# Autodesk Inventor assembly: Y-Carriage_LM3037
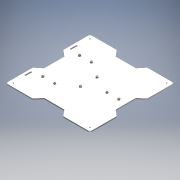
[picture p0: Inventor's stored thumbnail of the model, 180x180]
Saved by Autodesk Inventor 2020.2 (Build 242310000, 310)
## iProperties
Created: 2020-04-10
Part Number: Y-Carriage_LM3037
Document SubType Name: Assembly
Designer: rah75
Author: rah75
## Documents named in this file (10)
- C:\Users\rah75\Documents\GitHub\LETU-Maker\CAD\Autodesk Inventor\Base_3001-5999\Y-Carriage\Assemblies\Y-Carriage_LM3037.iam
- C:\Users\rah75\Documents\GitHub\LETU-Maker\CAD\Autodesk Inventor\Base_3001-5999\Y-Carriage\Fabricated_Parts\Y-Carriage_Plate_LM3033.ipt
- C:\Users\rah75\Documents\GitHub\LETU-Maker\CAD\Autodesk Inventor\Base_3001-5999\Y-Carriage\Printed_Parts\Y-Carriage_Belt_Mount_LM3035.ipt
- C:\Users\rah75\Documents\GitHub\LETU-Maker\CAD\Autodesk Inventor\Base_3001-5999\Y-Carriage\Printed_Parts\Y-Carriage_Belt_Clamp_LM3036.ipt
- C:\Users\rah75\Documents\GitHub\LETU-Maker\CAD\Autodesk Inventor\Base_3001-5999\Y-Carriage\Printed_Parts\Y-Carriage_Bearing_Mount_LM3034.ipt
- C:\Users\rah75\Documents\GitHub\LETU-Maker\CAD\Autodesk Inventor\Stock_Components_1001-2999\Fasteners\Nuts\heat_insert_m3_LM1017.ipt
- C:\Users\rah75\Documents\GitHub\LETU-Maker\CAD\Autodesk Inventor\Stock_Components_1001-2999\Power_Transmission\Bearings\linear_bearing_8x15mm_LM1031.ipt
- C:\Users\rah75\Documents\GitHub\LETU-Maker\CAD\Autodesk Inventor\Stock_Components_1001-2999\Fasteners\Screws\SHCS_m3x10_LM1015.ipt
- C:\Users\rah75\Documents\GitHub\LETU-Maker\CAD\Autodesk Inventor\Stock_Components_1001-2999\Fasteners\Washers_Spacers\washer_m3_LM1001.ipt
- C:\Users\rah75\Documents\GitHub\LETU-Maker\CAD\Autodesk Inventor\Stock_Components_1001-2999\Fasteners\Nuts\hex_nut_m3_LM1019.ipt
## Components (46 placed, 9 different names)
1. Y-Carriage_Plate_LM3033:1 — Insert:1, Insert:2, Insert:3, Insert:10, Mate:1, Insert:28, Insert:29, Insert:30, Insert:31, Insert:32, Insert:33, Insert:34, Insert:35
2. Y-Carriage_Belt_Mount_LM3035:1 — Insert:4, Insert:5, Insert:6, Insert:7, Insert:8, Insert:9
3. Y-Carriage_Belt_Clamp_LM3036:1 — Insert:12, Mate:3, Insert:36, Insert:37
4. Y-Carriage_Bearing_Mount_LM3034:1 — Insert:2, Insert:13, Insert:44, Insert:45
5. Y-Carriage_Bearing_Mount_LM3034:2 — Insert:3, Insert:15, Insert:40, Insert:41
6. Y-Carriage_Bearing_Mount_LM3034:3 — Insert:1, Insert:14, Insert:42, Insert:43
7. Y-Carriage_Belt_Clamp_LM3036:2 — Insert:11, Mate:2, Insert:38, Insert:39
8. heat_insert_m3_LM1017:1 — Insert:7, Insert:12
9. heat_insert_m3_LM1017:2 — Insert:5, Mate:2
10. heat_insert_m3_LM1017:3 — Insert:6, Mate:3
11. heat_insert_m3_LM1017:4 — Insert:9, Mate:1
12. heat_insert_m3_LM1017:5 — Insert:4, Insert:11
13. heat_insert_m3_LM1017:6 — Insert:8, Insert:10
14. linear_bearing_8x15mm_LM1031:1 — Insert:15
15. linear_bearing_8x15mm_LM1031:2 — Insert:14
16. linear_bearing_8x15mm_LM1031:3 — Insert:13
17. SHCS_m3x10_LM1015:1 — Insert:19
18. SHCS_m3x10_LM1015:2 — Insert:24
19. SHCS_m3x10_LM1015:3 — Insert:23
20. SHCS_m3x10_LM1015:4 — Insert:22
21. SHCS_m3x10_LM1015:5 — Insert:17
22. SHCS_m3x10_LM1015:6 — Insert:18
23. SHCS_m3x10_LM1015:7 — Insert:16
24. SHCS_m3x10_LM1015:8 — Insert:20
25. SHCS_m3x10_LM1015:9 — Insert:21
26. SHCS_m3x10_LM1015:10 — Insert:27
27. SHCS_m3x10_LM1015:11 — Insert:26
28. SHCS_m3x10_LM1015:12 — Insert:25
29. washer_m3_LM1001:1 — Insert:21, Insert:33
30. washer_m3_LM1001:2 — Insert:18, Insert:37
31. washer_m3_LM1001:3 — Insert:20, Insert:34
32. washer_m3_LM1001:4 — Insert:22, Insert:32
33. washer_m3_LM1001:5 — Insert:27, Insert:28
34. washer_m3_LM1001:6 — Insert:26, Insert:35
35. washer_m3_LM1001:7 — Insert:23, Insert:38
36. washer_m3_LM1001:8 — Insert:25, Insert:39
37. washer_m3_LM1001:9 — Insert:24, Insert:29
38. washer_m3_LM1001:10 — Insert:19, Insert:30
39. washer_m3_LM1001:11 — Insert:17, Insert:31
40. washer_m3_LM1001:12 — Insert:16, Insert:36
41. hex_nut_m3_LM1019:1 — Insert:40
42. hex_nut_m3_LM1019:2 — Insert:43
43. hex_nut_m3_LM1019:3 — Insert:44
44. hex_nut_m3_LM1019:4 — Insert:45
45. hex_nut_m3_LM1019:5 — Insert:42
46. hex_nut_m3_LM1019:6 — Insert:41
## Relationships (48: Insert 45, Mate 3)
- Insert:1: Y-Carriage_Plate_LM3033:1 ↔ Y-Carriage_Bearing_Mount_LM3034:3
- Insert:2: Y-Carriage_Plate_LM3033:1 ↔ Y-Carriage_Bearing_Mount_LM3034:1
- Insert:3: Y-Carriage_Plate_LM3033:1 ↔ Y-Carriage_Bearing_Mount_LM3034:2
- Insert:4: Y-Carriage_Belt_Mount_LM3035:1 ↔ heat_insert_m3_LM1017:5
- Insert:5: Y-Carriage_Belt_Mount_LM3035:1 ↔ heat_insert_m3_LM1017:2
- Insert:6: Y-Carriage_Belt_Mount_LM3035:1 ↔ heat_insert_m3_LM1017:3
- Insert:7: Y-Carriage_Belt_Mount_LM3035:1 ↔ heat_insert_m3_LM1017:1
- Insert:8: Y-Carriage_Belt_Mount_LM3035:1 ↔ heat_insert_m3_LM1017:6
- Insert:9: Y-Carriage_Belt_Mount_LM3035:1 ↔ heat_insert_m3_LM1017:4
- Insert:10: Y-Carriage_Plate_LM3033:1 ↔ heat_insert_m3_LM1017:6
- Mate:1: Y-Carriage_Plate_LM3033:1 ↔ heat_insert_m3_LM1017:4
- Insert:11: Y-Carriage_Belt_Clamp_LM3036:2 ↔ heat_insert_m3_LM1017:5
- Insert:12: Y-Carriage_Belt_Clamp_LM3036:1 ↔ heat_insert_m3_LM1017:1
- Mate:2: Y-Carriage_Belt_Clamp_LM3036:2 ↔ heat_insert_m3_LM1017:2
- Mate:3: Y-Carriage_Belt_Clamp_LM3036:1 ↔ heat_insert_m3_LM1017:3
- Insert:13: Y-Carriage_Bearing_Mount_LM3034:1 ↔ linear_bearing_8x15mm_LM1031:3
- Insert:14: Y-Carriage_Bearing_Mount_LM3034:3 ↔ linear_bearing_8x15mm_LM1031:2
- Insert:15: Y-Carriage_Bearing_Mount_LM3034:2 ↔ linear_bearing_8x15mm_LM1031:1
- Insert:16: SHCS_m3x10_LM1015:7 ↔ washer_m3_LM1001:12
- Insert:17: SHCS_m3x10_LM1015:5 ↔ washer_m3_LM1001:11
- Insert:18: SHCS_m3x10_LM1015:6 ↔ washer_m3_LM1001:2
- Insert:19: SHCS_m3x10_LM1015:1 ↔ washer_m3_LM1001:10
- Insert:20: SHCS_m3x10_LM1015:8 ↔ washer_m3_LM1001:3
- Insert:21: SHCS_m3x10_LM1015:9 ↔ washer_m3_LM1001:1
- Insert:22: SHCS_m3x10_LM1015:4 ↔ washer_m3_LM1001:4
- Insert:23: SHCS_m3x10_LM1015:3 ↔ washer_m3_LM1001:7
- Insert:24: SHCS_m3x10_LM1015:2 ↔ washer_m3_LM1001:9
- Insert:25: SHCS_m3x10_LM1015:12 ↔ washer_m3_LM1001:8
- Insert:26: SHCS_m3x10_LM1015:11 ↔ washer_m3_LM1001:6
- Insert:27: SHCS_m3x10_LM1015:10 ↔ washer_m3_LM1001:5
- Insert:28: Y-Carriage_Plate_LM3033:1 ↔ washer_m3_LM1001:5
- Insert:29: Y-Carriage_Plate_LM3033:1 ↔ washer_m3_LM1001:9
- Insert:30: Y-Carriage_Plate_LM3033:1 ↔ washer_m3_LM1001:10
- Insert:31: Y-Carriage_Plate_LM3033:1 ↔ washer_m3_LM1001:11
- Insert:32: Y-Carriage_Plate_LM3033:1 ↔ washer_m3_LM1001:4
- Insert:33: Y-Carriage_Plate_LM3033:1 ↔ washer_m3_LM1001:1
- Insert:34: Y-Carriage_Plate_LM3033:1 ↔ washer_m3_LM1001:3
- Insert:35: Y-Carriage_Plate_LM3033:1 ↔ washer_m3_LM1001:6
- Insert:36: Y-Carriage_Belt_Clamp_LM3036:1 ↔ washer_m3_LM1001:12
- Insert:37: Y-Carriage_Belt_Clamp_LM3036:1 ↔ washer_m3_LM1001:2
- Insert:38: Y-Carriage_Belt_Clamp_LM3036:2 ↔ washer_m3_LM1001:7
- Insert:39: Y-Carriage_Belt_Clamp_LM3036:2 ↔ washer_m3_LM1001:8
- Insert:40: Y-Carriage_Bearing_Mount_LM3034:2 ↔ hex_nut_m3_LM1019:1
- Insert:41: Y-Carriage_Bearing_Mount_LM3034:2 ↔ hex_nut_m3_LM1019:6
- Insert:42: Y-Carriage_Bearing_Mount_LM3034:3 ↔ hex_nut_m3_LM1019:5
- Insert:43: Y-Carriage_Bearing_Mount_LM3034:3 ↔ hex_nut_m3_LM1019:2
- Insert:44: Y-Carriage_Bearing_Mount_LM3034:1 ↔ hex_nut_m3_LM1019:3
- Insert:45: Y-Carriage_Bearing_Mount_LM3034:1 ↔ hex_nut_m3_LM1019:4
